# Autodesk Inventor assembly: trapezoid ramp assembly
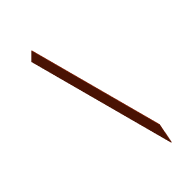
[picture p0: Inventor's stored thumbnail of the model, 180x180]
Saved by Autodesk Inventor 2015 (Build 190159000, 159)
## iProperties
Created: 2015-01-20
Part Number: trapezoid ramp assembly
Document SubType Name: Assembly
Designer: Peter
Author: Peter
## Documents named in this file (3)
- T:\FILES\FIRST-Team-1719-CAD-Team\2015 Playing Field\Team 1719 Practice Field\Scoring Platform - Construction Design\trapezoid ramp assembly.iam
- T:\FILES\FIRST-Team-1719-CAD-Team\2015 Playing Field\Team 1719 Practice Field\Scoring Platform - Construction Design\trapezoid polycarbonate ramp 125.ipt
- T:\FILES\FIRST-Team-1719-CAD-Team\2015 Playing Field\Team 1719 Practice Field\Scoring Platform - Construction Design\trapezoid plywood ramp 375.ipt
## Components (2 placed, 2 different names)
1. trapezoid polycarbonate ramp 125:1 — Mate:1, Flush:1
2. trapezoid plywood ramp 375:1 — Mate:1, Flush:1
## Relationships (2: Mate 1, Flush 1)
- Mate:1: trapezoid polycarbonate ramp 125:1 ↔ trapezoid plywood ramp 375:1
- Flush:1: trapezoid polycarbonate ramp 125:1 ↔ trapezoid plywood ramp 375:1
